# Autodesk Inventor assembly: bearing holder w bearing (treadmill)
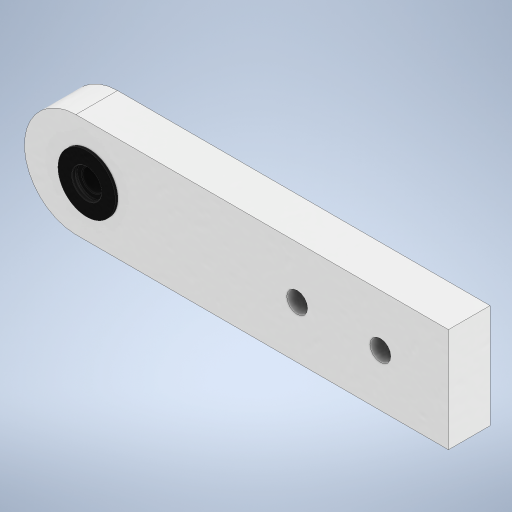
[picture p0: Inventor's stored thumbnail of the model, 512x512]
Saved by Autodesk Inventor 2024 (Build 280153000, 153)
## iProperties
Created: 2023-02-06
Part Number: bearing holder w bearing (treadmill)
Document SubType Name: Assembly
Designer: rosam
Author: rosam
## Documents named in this file (3)
- C:\Users\rosam\OneDrive\Documents\github_latest\Hardware\Tablet-Rig\Assemblies\bearing holder w bearing (treadmill).iam
- C:\Users\rosam\OneDrive\Documents\github_latest\Hardware\Tablet-Rig\parts\bearing holder (treadmill).ipt
- C:\Users\rosam\OneDrive\Documents\github_latest\Hardware\Tablet-Rig\parts\McMaster_Bearings\1293N105_Self-Aligning Flanged Ball Bearing.ipt
## Components (2 placed, 2 different names)
1. bearing holder (treadmill):1 — Mate:1, Mate:2
2. 1293N105_Self-Aligning Flanged Ball Bearing:1 — Mate:1, Mate:2
## Relationships (2: Mate 2)
- Mate:1: bearing holder (treadmill):1 ↔ 1293N105_Self-Aligning Flanged Ball Bearing:1
- Mate:2: bearing holder (treadmill):1 ↔ 1293N105_Self-Aligning Flanged Ball Bearing:1
